# Autodesk Inventor assembly: inner_MIR
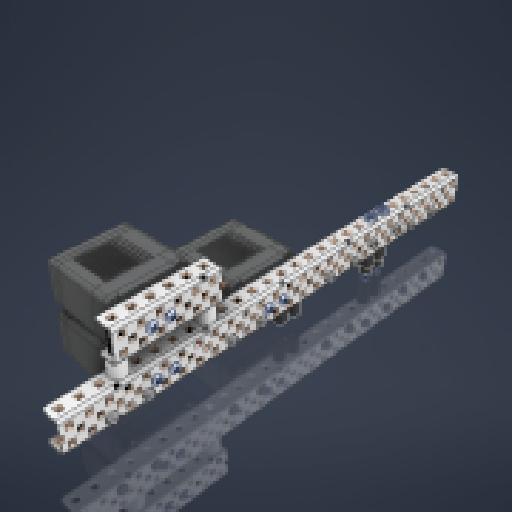
[picture p0: Inventor's stored thumbnail of the model, 512x512]
Saved by Autodesk Inventor 2024 (Build 280153000, 153)
## iProperties
Created: 2023-10-18
Part Number: inner_MIR
Document SubType Name: Assembly
Designer: Averey Ku
Author: Averey Ku
## Documents named in this file (17)
- D:\vex_robotics\hardware\cad\goated_v0.1\chassis\mirrored_parts\inner_MIR.iam
- D:\vex_robotics\hardware\cad\goated_v0.1\chassis\mirrored_parts\Alu C 1x2x1x28_MIR.ipt
- D:\vex_robotics\hardware\cad\goated_v0.1\chassis\mirrored_parts\Alu C 1x2x1x6_MIR.ipt
- D:\vex_robotics\hardware\cad\VEX-CAD-Inventor-1.41\Structure\Standoff\Standoff .875.ipt
- D:\vex_robotics\hardware\cad\VEX-CAD-Inventor-1.41\Structure\Standoff.ipt
- D:\vex_robotics\hardware\cad\goated_v0.1\chassis\mirrored_parts\.375 OD Aluminum Spacer 0.875_MIR.ipt
- D:\vex_robotics\hardware\cad\goated_v0.1\chassis\mirrored_parts\SteelM-StarS_MIR.iam
- D:\vex_robotics\hardware\cad\VEX-CAD-Inventor-1.41\Motion\Spacers\Spacer Nylon .500 OD\NSpacer White .500 OD x .500.ipt
- D:\vex_robotics\hardware\cad\VEX-CAD-Inventor-1.41\Motion\Spacers\Spacer Nylon .500 OD.ipt
- D:\vex_robotics\hardware\cad\goated_v0.1\chassis\mirrored_parts\lightweight_bearing_MIR.iam
- D:\vex_robotics\hardware\cad\VEX-CAD-Inventor-1.41\Motion\Spacers\Spacer Nylon .375 OD\NSpacer .375 OD x .500.ipt
- D:\vex_robotics\hardware\cad\VEX-CAD-Inventor-1.41\Motion\Spacers\Spacer Nylon .375 OD.ipt
- D:\vex_robotics\hardware\cad\goated_v0.1\chassis\mirrored_parts\Nut Keps_MIR.ipt
- D:\vex_robotics\hardware\cad\VEX-CAD-Inventor-1.41\Structure\Hardware\Screw Shoulder Robosource\SScrew Shoulder Smooth 2.000 x .04.ipt
- D:\vex_robotics\hardware\cad\VEX-CAD-Inventor-1.41\Structure\Hardware\Screw Shoulder Robosource.ipt
- D:\vex_robotics\hardware\cad\goated_v0.1\chassis\mirrored_parts\Nut Hex_MIR.ipt
- D:\vex_robotics\hardware\cad\VEX-CAD-Inventor-1.41\Motion\Spacers\Spacer Nylon .375 OD\NSpacer .375 OD x .250.ipt
## Components (35 placed, 12 different names)
1. Alu C 1x2x1x28_MIR:1 — Mate:1, Insert:3, Insert:4, Mate:3, Insert:6, Insert:8, Insert:7, Mate:4, Insert:9, Mate:5, Insert:10, Mate:6, Insert:11, Mate:7, Insert:12, Insert:14, Insert:13, Insert:18, Insert:17, Insert:16, Insert:15, Insert:24, Mate:9, Insert:25, Mate:10, Insert:26, Insert:32, Insert:33, Insert:36, Insert:37
2. Alu C 1x2x1x6_MIR:1 — Mate:1, Insert:3, Insert:1, Insert:2, Mate:2, Insert:5
3. Standoff .875:1 — Insert:1
4. Standoff .875:2 — Insert:2
5. .375 OD Aluminum Spacer 0.875_MIR:1 — Insert:4
6. SteelM-StarS_MIR:1 [sub-assembly] — Mate:2, Insert:5
7. SteelM-StarS_MIR:2 [sub-assembly] — Mate:3, Insert:6
8. NSpacer White .500 OD x .500:1 — Insert:8
9. NSpacer White .500 OD x .500:2 — Insert:7
10. SteelM-StarS_MIR:3 [sub-assembly] — Mate:4, Insert:9
11. lightweight_bearing_MIR:1 [sub-assembly] — Mate:5, Insert:10, Insert:28
12. lightweight_bearing_MIR:2 [sub-assembly] — Mate:6, Insert:11, Insert:29
13. lightweight_bearing_MIR:3 [sub-assembly] — Mate:7, Insert:12, Insert:27
14. NSpacer .375 OD x .500:1 — Insert:14, Insert:21, Insert:34
15. NSpacer .375 OD x .500:2 — Insert:13, Insert:20, Insert:35
16. Nut Keps_MIR:1 — Insert:18
17. Nut Keps_MIR:2 — Insert:17
18. Nut Keps_MIR:3 — Insert:16
19. Nut Keps_MIR:4 — Insert:15
20. SScrew Shoulder Smooth 2.000 x .04:1 — Insert:20
21. SScrew Shoulder Smooth 2.000 x .04:2 — Insert:21
22. Nut Hex_MIR:1 — Insert:36
23. Nut Hex_MIR:2 — Insert:37
24. .375 OD Aluminum Spacer 0.875_MIR:2 — Insert:24
25. lightweight_bearing_MIR:4 [sub-assembly] — Mate:9, Insert:25, Insert:30
26. lightweight_bearing_MIR:5 [sub-assembly] — Mate:10, Insert:26, Insert:31
27. Nut Hex_MIR:3 — Insert:27
28. Nut Hex_MIR:4 — Insert:29
29. Nut Hex_MIR:5 — Insert:31
30. Nut Hex_MIR:6 — Insert:30
31. Nut Hex_MIR:7 — Insert:28
32. NSpacer .375 OD x .500:3 — Insert:32
33. NSpacer .375 OD x .500:4 — Insert:33
34. NSpacer .375 OD x .250:5 — Insert:35
35. NSpacer .375 OD x .250:6 — Insert:34
## Relationships (43: Insert 34, Mate 9)
- Mate:1: Alu C 1x2x1x28_MIR:1 ↔ Alu C 1x2x1x6_MIR:1
- Insert:3 (12.7 mm): Alu C 1x2x1x28_MIR:1 ↔ Alu C 1x2x1x6_MIR:1
- Insert:1: Alu C 1x2x1x6_MIR:1 ↔ Standoff .875:1
- Insert:2: Alu C 1x2x1x6_MIR:1 ↔ Standoff .875:2
- Insert:4: Alu C 1x2x1x28_MIR:1 ↔ .375 OD Aluminum Spacer 0.875_MIR:1
- Mate:2: Alu C 1x2x1x6_MIR:1 ↔ SteelM-StarS_MIR:1
- Insert:5: Alu C 1x2x1x6_MIR:1 ↔ SteelM-StarS_MIR:1
- Mate:3: Alu C 1x2x1x28_MIR:1 ↔ SteelM-StarS_MIR:2
- Insert:6: Alu C 1x2x1x28_MIR:1 ↔ SteelM-StarS_MIR:2
- Insert:8: Alu C 1x2x1x28_MIR:1 ↔ NSpacer White .500 OD x .500:1
- Insert:7: Alu C 1x2x1x28_MIR:1 ↔ NSpacer White .500 OD x .500:2
- Mate:4: Alu C 1x2x1x28_MIR:1 ↔ SteelM-StarS_MIR:3
- Insert:9: Alu C 1x2x1x28_MIR:1 ↔ SteelM-StarS_MIR:3
- Mate:5: Alu C 1x2x1x28_MIR:1 ↔ lightweight_bearing_MIR:1
- Insert:10: Alu C 1x2x1x28_MIR:1 ↔ lightweight_bearing_MIR:1
- Mate:6: Alu C 1x2x1x28_MIR:1 ↔ lightweight_bearing_MIR:2
- Insert:11: Alu C 1x2x1x28_MIR:1 ↔ lightweight_bearing_MIR:2
- Mate:7: Alu C 1x2x1x28_MIR:1 ↔ lightweight_bearing_MIR:3
- Insert:12: Alu C 1x2x1x28_MIR:1 ↔ lightweight_bearing_MIR:3
- Insert:14: Alu C 1x2x1x28_MIR:1 ↔ NSpacer .375 OD x .500:1
- Insert:13: Alu C 1x2x1x28_MIR:1 ↔ NSpacer .375 OD x .500:2
- Insert:18: Alu C 1x2x1x28_MIR:1 ↔ Nut Keps_MIR:1
- Insert:17: Alu C 1x2x1x28_MIR:1 ↔ Nut Keps_MIR:2
- Insert:16: Alu C 1x2x1x28_MIR:1 ↔ Nut Keps_MIR:3
- Insert:15: Alu C 1x2x1x28_MIR:1 ↔ Nut Keps_MIR:4
- Insert:20 (7.9375 mm): NSpacer .375 OD x .500:2 ↔ SScrew Shoulder Smooth 2.000 x .04:1
- Insert:21 (7.9375 mm): NSpacer .375 OD x .500:1 ↔ SScrew Shoulder Smooth 2.000 x .04:2
- Insert:24: Alu C 1x2x1x28_MIR:1 ↔ .375 OD Aluminum Spacer 0.875_MIR:2
- Mate:9: Alu C 1x2x1x28_MIR:1 ↔ lightweight_bearing_MIR:4
- Insert:25: Alu C 1x2x1x28_MIR:1 ↔ lightweight_bearing_MIR:4
- Mate:10: Alu C 1x2x1x28_MIR:1 ↔ lightweight_bearing_MIR:5
- Insert:26: Alu C 1x2x1x28_MIR:1 ↔ lightweight_bearing_MIR:5
- Insert:27 (1.27 mm): lightweight_bearing_MIR:3 ↔ Nut Hex_MIR:3
- Insert:29 (1.27 mm): lightweight_bearing_MIR:2 ↔ Nut Hex_MIR:4
- Insert:31 (1.27 mm): lightweight_bearing_MIR:5 ↔ Nut Hex_MIR:5
- Insert:30 (1.27 mm): lightweight_bearing_MIR:4 ↔ Nut Hex_MIR:6
- Insert:28 (1.27 mm): lightweight_bearing_MIR:1 ↔ Nut Hex_MIR:7
- Insert:32: Alu C 1x2x1x28_MIR:1 ↔ NSpacer .375 OD x .500:3
- Insert:33: Alu C 1x2x1x28_MIR:1 ↔ NSpacer .375 OD x .500:4
- Insert:34: NSpacer .375 OD x .500:1 ↔ NSpacer .375 OD x .250:6
- Insert:35: NSpacer .375 OD x .500:2 ↔ NSpacer .375 OD x .250:5
- Insert:36: Alu C 1x2x1x28_MIR:1 ↔ Nut Hex_MIR:1
- Insert:37: Alu C 1x2x1x28_MIR:1 ↔ Nut Hex_MIR:2
